# Autodesk Inventor assembly: 頭_1_2
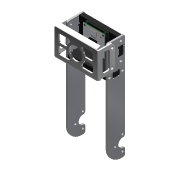
[picture p0: Inventor's stored thumbnail of the model, 180x180]
Saved by Autodesk Inventor 2017.3 (Build 213256000, 256)
## iProperties
Created: 2016-05-10
Part Number: 頭_1_2
Document SubType Name: Assembly
Designer: hiroaki
Mass: 19.311 g
Surface Area: 122.669 cm^2
Volume: 8.04943 cm^3
Density: 2.39905 g/cm^3
Author: hiroaki
## Documents named in this file (7)
- C:\Users\haya\Desktop\差分\171119OpenPlatform_設計\OpenPlatform ver.1.0\上半身\頭\頭_1_2.iam
- C:\Users\haya\Desktop\差分\171119OpenPlatform_設計\OpenPlatform ver.1.0\インポートされたコンポーネント\RasPi_Camera\RasPi_Camera.iam
- C:\Users\haya\Desktop\差分\171119OpenPlatform_設計\OpenPlatform ver.1.0\上半身\頭\頭_メインフレーム_1_3.ipt
- C:\Users\haya\Desktop\差分\171119OpenPlatform_設計\OpenPlatform ver.1.0\上半身\頭\頭_メインフレーム_1_4.ipt
- C:\Users\haya\Desktop\差分\171119OpenPlatform_設計\OpenPlatform ver.1.0\上半身\頭\頭_メインサイドフレーム.ipt
- C:\Users\haya\Desktop\差分\171119OpenPlatform_設計\OpenPlatform ver.1.0\上半身\頭\頭_メインフレームセンター.ipt
- C:\Users\haya\Desktop\差分\171119OpenPlatform_設計\OpenPlatform ver.1.0\上半身\頭\頭_メインフレームセンター２.ipt
## Components (7 placed, 6 different names)
1. RasPi_Camera:1 [sub-assembly] — 挿入:3, 挿入:4, 挿入:5
2. 頭_メインフレーム_1_3:1 — 挿入:3, 挿入:4, 挿入:5, 挿入:12, 挿入:13
3. 頭_メインフレーム_1_4:1 — 挿入:6, 挿入:7
4. 頭_メインサイドフレーム:1 — 挿入:6, 挿入:7, 挿入:8, 挿入:9, 挿入:14, 挿入:15
5. 頭_メインサイドフレーム:2 — 挿入:10, 挿入:11, 挿入:16, 挿入:17
6. 頭_メインフレームセンター:1 — 挿入:8, 挿入:9, 挿入:10, 挿入:11, 挿入:12, 挿入:13
7. 頭_メインフレームセンター２:1 — 挿入:14, 挿入:15, 挿入:16, 挿入:17
## Relationships (15: Insert 15)
- 挿入:3 [Insert]: RasPi_Camera:1 ↔ 頭_メインフレーム_1_3:1
- 挿入:4 [Insert]: RasPi_Camera:1 ↔ 頭_メインフレーム_1_3:1
- 挿入:5 [Insert]: RasPi_Camera:1 ↔ 頭_メインフレーム_1_3:1
- 挿入:6 [Insert]: 頭_メインフレーム_1_4:1 ↔ 頭_メインサイドフレーム:1
- 挿入:7 [Insert]: 頭_メインフレーム_1_4:1 ↔ 頭_メインサイドフレーム:1
- 挿入:8 [Insert]: 頭_メインサイドフレーム:1 ↔ 頭_メインフレームセンター:1
- 挿入:9 [Insert]: 頭_メインサイドフレーム:1 ↔ 頭_メインフレームセンター:1
- 挿入:10 [Insert]: 頭_メインサイドフレーム:2 ↔ 頭_メインフレームセンター:1
- 挿入:11 [Insert]: 頭_メインサイドフレーム:2 ↔ 頭_メインフレームセンター:1
- 挿入:12 [Insert]: 頭_メインフレーム_1_3:1 ↔ 頭_メインフレームセンター:1
- 挿入:13 [Insert]: 頭_メインフレーム_1_3:1 ↔ 頭_メインフレームセンター:1
- 挿入:14 [Insert]: 頭_メインサイドフレーム:1 ↔ 頭_メインフレームセンター２:1
- 挿入:15 [Insert]: 頭_メインサイドフレーム:1 ↔ 頭_メインフレームセンター２:1
- 挿入:16 [Insert]: 頭_メインサイドフレーム:2 ↔ 頭_メインフレームセンター２:1
- 挿入:17 [Insert]: 頭_メインサイドフレーム:2 ↔ 頭_メインフレームセンター２:1
